# Autodesk Inventor assembly: vehicle assembly v2
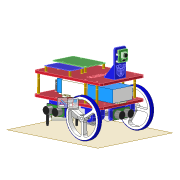
[picture p0: Inventor's stored thumbnail of the model, 180x180]
Saved by Autodesk Inventor 2022 (Build 260153000, 153)
## iProperties
Created: 2024-06-06
Part Number: vehicle assembly v2
Document SubType Name: Assembly
Designer: david
Author: david
## Documents named in this file (29)
- C:\Users\david\OneDrive\Documents\Singapore Polytechnic\SP-RITE\WRO FE 2024 (Repository)\models\vehicle 3D model\vehicle assembly v2.iam
- C:\Users\david\OneDrive\Documents\Singapore Polytechnic\SP-RITE\WRO FE 2024 (Repository)\models\vehicle 3D model\base plate.ipt
- C:\Users\david\OneDrive\Documents\Singapore Polytechnic\SP-RITE\WRO FE 2024 (Repository)\models\vehicle 3D model\bearing holder.ipt
- C:\Users\david\OneDrive\Documents\Singapore Polytechnic\SP-RITE\WRO FE 2024 (Repository)\models\vehicle 3D model\servo motor HS-7955TG.iam
- C:\Users\david\OneDrive\Documents\Singapore Polytechnic\SP-RITE\WRO FE 2024 (Repository)\models\vehicle 3D model\steering top half.ipt
- steering top half.ipt
- C:\Users\david\OneDrive\Documents\Singapore Polytechnic\SP-RITE\WRO FE 2024 (Repository)\models\vehicle 3D model\dfifferential.ipt
- C:\Users\david\OneDrive\Documents\Singapore Polytechnic\SP-RITE\WRO FE 2024 (Repository)\models\vehicle 3D model\front wheel.ipt
- C:\Users\david\OneDrive\Documents\Singapore Polytechnic\SP-RITE\WRO FE 2024 (Repository)\models\vehicle 3D model\rear wheel 86mm.ipt
- C:\Users\david\OneDrive\Documents\Singapore Polytechnic\SP-RITE\WRO FE 2024 (Repository)\models\vehicle 3D model\rear shaft.ipt
- rear shaft.ipt
- C:\Users\david\OneDrive\Documents\Singapore Polytechnic\SP-RITE\WRO FE 2024 (Repository)\models\vehicle 3D model\12v DC motor.ipt
- C:\Users\david\OneDrive\Documents\Singapore Polytechnic\SP-RITE\WRO FE 2024 (Repository)\models\vehicle 3D model\stand M3-L10.ipt
- C:\Users\david\OneDrive\Documents\Singapore Polytechnic\SP-RITE\WRO FE 2024 (Repository)\models\vehicle 3D model\top plate.ipt
- C:\Users\david\OneDrive\Documents\Singapore Polytechnic\SP-RITE\WRO FE 2024 (Repository)\models\vehicle 3D model\raspberry pi.ipt
- C:\Users\david\OneDrive\Documents\Singapore Polytechnic\SP-RITE\WRO FE 2024 (Repository)\models\vehicle 3D model\3s lipo battery.ipt
- C:\Users\david\OneDrive\Documents\Singapore Polytechnic\SP-RITE\WRO FE 2024 (Repository)\models\vehicle 3D model\ultrasonic mount.ipt
- C:\Users\david\OneDrive\Documents\Singapore Polytechnic\SP-RITE\WRO FE 2024 (Repository)\models\vehicle 3D model\US-015.ipt
- C:\Users\david\OneDrive\Documents\Singapore Polytechnic\SP-RITE\WRO FE 2024 (Repository)\models\vehicle 3D model\stand M3-L30.ipt
- C:\Users\david\OneDrive\Documents\Singapore Polytechnic\SP-RITE\WRO FE 2024 (Repository)\models\vehicle 3D model\LM2596 Buck Converter.ipt
- C:\Users\david\OneDrive\Documents\Singapore Polytechnic\SP-RITE\WRO FE 2024 (Repository)\models\vehicle 3D model\camera mount.ipt
- C:\Users\david\OneDrive\Documents\Singapore Polytechnic\SP-RITE\WRO FE 2024 (Repository)\models\vehicle 3D model\raspberry pi camera.ipt
- C:\Users\david\OneDrive\Documents\Singapore Polytechnic\SP-RITE\WRO FE 2024 (Repository)\models\vehicle 3D model\stub.ipt
- C:\Users\david\OneDrive\Documents\Singapore Polytechnic\SP-RITE\WRO FE 2024 (Repository)\models\vehicle 3D model\front shaft.ipt
- C:\Users\david\OneDrive\Documents\Singapore Polytechnic\SP-RITE\WRO FE 2024 (Repository)\models\vehicle 3D model\steering bottom half.ipt
- C:\Users\david\OneDrive\Documents\Singapore Polytechnic\SP-RITE\WRO FE 2024 (Repository)\models\vehicle 3D model\driver gear adapter v2.ipt
- C:\Users\david\OneDrive\Documents\Singapore Polytechnic\SP-RITE\WRO FE 2024 (Repository)\models\vehicle 3D model\ultrasonic mount (front) v2.ipt
- C:\Users\david\OneDrive\Documents\Singapore Polytechnic\SP-RITE\WRO FE 2024 (Repository)\models\vehicle 3D model\3S lipo holder v2.ipt
- C:\Users\david\OneDrive\Documents\Singapore Polytechnic\SP-RITE\WRO FE 2024 (Repository)\models\vehicle 3D model\12v DC motor mount v2.ipt
## Components (56 placed, 26 different names)
1. base plate:1 — Insert:60, Insert:61, Insert:62, Insert:63, Mate:9, Mate:10, Mate:11, Flush:6, Flush:7, Flush:8, Insert:74, Insert:75, Insert:134, Insert:135, Insert:136, Insert:137, Insert:138, Insert:139, Insert:140, Insert:141, Insert:196, Insert:197, Insert:198, Insert:199, Insert:200, Insert:201, Insert:202, Insert:203, Mate:19, Insert:208, Insert:209
2. top plate:1 — Insert:153, Insert:175, Insert:176, Insert:177, Insert:186, Insert:187, Insert:188, Insert:189, Insert:190, Insert:191
3. bearing holder:1 — Insert:134, Insert:135, Insert:143
4. bearing holder:2 — Insert:136, Insert:137
5. bearing holder:3 — Insert:140, Insert:141
6. bearing holder:4 — Insert:138, Insert:139, Insert:142
7. dfifferential:1 — Mate:16, Flush:10
8. rear shaft:1 — Insert:83, Angle:9, Insert:143, Mate:16
9. rear shaft:2 — Angle:8, Insert:142, Insert:205
10. rear wheel 86mm:1 — Insert:83, Angle:9
11. rear wheel 86mm:2 — Tangent:1, Angle:8, Insert:205
12. 12v DC motor:1 — Angle:14, Insert:204, Insert:206, Insert:207
13. servo motor HS-7955TG:1 [sub-assembly] — Mate:2, Insert:20, Mate:9, Mate:10, Mate:11
14. steering top half:1 — Insert:20, Mate:14, Mate:15, Angle:12, Angle:13
15. steering bottom half:1 — Mate:14, Mate:15, Angle:12, Insert:166
16. front wheel:1 — Insert:164, Angle:10
17. front wheel:2 — Insert:165, Angle:11
18. stand M3-L30:2 — Insert:60, Insert:150
19. stand M3-L30:3 — Insert:63, Insert:146
20. stand M3-L30:1 — Insert:61, Insert:151
21. stand M3-L30:4 — Insert:62, Insert:148
22. stand M3-L30:9 — Insert:74, Insert:149
23. stand M3-L30:10 — Insert:75, Insert:147
24. stand M3-L10:1 — Insert:169, Insert:191
25. stand M3-L10:2 — Insert:168, Insert:189
26. stand M3-L10:3 — Insert:59
27. stand M3-L10:4 — Insert:58
28. 3s lipo battery:1 — Flush:9, Mate:18, Flush:11
29. ultrasonic mount:1 — Insert:102, Insert:103, Insert:200, Insert:201
30. ultrasonic mount:2 — Insert:106, Insert:107, Insert:198, Insert:199
31. US-015:1 — Insert:102, Insert:103
32. US-015:2 — Insert:106, Insert:107
33. US-015:3 — Insert:194, Insert:195
34. LM2596 Buck Converter:1 — Insert:112, Insert:113, Insert:169, Insert:170
35. stand M3-L10:5 — Insert:167, Insert:188
36. stand M3-L10:6 — Insert:170, Insert:190
37. stand M3-L10:7 — Insert:112
38. stand M3-L10:8 — Insert:113
39. raspberry pi:1 — Insert:58, Insert:59, Insert:167, Insert:168
40. camera mount:1 — Insert:124, Insert:125, Insert:186, Insert:187
41. raspberry pi camera:1 — Insert:120, Insert:121, Insert:122, Insert:123
42. stub:1 — Insert:123
43. stub:2 — Insert:121, Insert:124
44. stub:3 — Insert:122
45. stub:4 — Insert:120, Insert:125
46. stand M3-L10:9 — Insert:148, Insert:177
47. stand M3-L10:10 — Insert:147
48. stand M3-L10:11 — Insert:151, Insert:153
49. stand M3-L10:12 — Insert:150, Insert:175
50. stand M3-L10:13 — Insert:149
51. stand M3-L10:14 — Insert:146, Insert:176
52. front shaft — Insert:164, Angle:10, Insert:165, Angle:11, Insert:166
53. driver gear adapter v2:1 — Angle:14, Insert:204
54. ultrasonic mount (front) v2:1 — Insert:194, Insert:195, Insert:196, Insert:197
55. 3S lipo holder v2:1 — Insert:202, Insert:203, Mate:18, Flush:11
56. 12v DC motor mount v2:1 — Mate:19, Insert:206, Insert:207, Insert:208, Insert:209
## Relationships (95: Insert 71, Mate 9, Angle 8, Flush 6, Tangent 1)
- Mate:2: servo motor HS-7955TG:1
- Insert:20: servo motor HS-7955TG:1 ↔ steering top half:1
- Angle:4 (0 deg)
- Tangent:1: rear wheel 86mm:2
- Insert:58: stand M3-L10:4 ↔ raspberry pi:1
- Insert:59: stand M3-L10:3 ↔ raspberry pi:1
- Insert:60: base plate:1 ↔ stand M3-L30:2
- Insert:61: base plate:1 ↔ stand M3-L30:1
- Insert:62: base plate:1 ↔ stand M3-L30:4
- Insert:63: base plate:1 ↔ stand M3-L30:3
- Mate:9: base plate:1 ↔ servo motor HS-7955TG:1
- Mate:10: base plate:1 ↔ servo motor HS-7955TG:1
- Mate:11: base plate:1 ↔ servo motor HS-7955TG:1
- Flush:6: base plate:1
- Flush:7: base plate:1
- Flush:8: base plate:1
- Insert:74: base plate:1 ↔ stand M3-L30:9
- Insert:75: base plate:1 ↔ stand M3-L30:10
- Insert:83: rear shaft:1 ↔ rear wheel 86mm:1
- Angle:8 (180 deg): rear shaft:2 ↔ rear wheel 86mm:2
- Angle:9 (180 deg): rear shaft:1 ↔ rear wheel 86mm:1
- Insert:102: ultrasonic mount:1 ↔ US-015:1
- Insert:103: ultrasonic mount:1 ↔ US-015:1
- Insert:106: ultrasonic mount:2 ↔ US-015:2
- Insert:107: ultrasonic mount:2 ↔ US-015:2
- Insert:112: LM2596 Buck Converter:1 ↔ stand M3-L10:7
- Insert:113: LM2596 Buck Converter:1 ↔ stand M3-L10:8
- Insert:120: raspberry pi camera:1 ↔ stub:4
- Insert:121: raspberry pi camera:1 ↔ stub:2
- Insert:122: raspberry pi camera:1 ↔ stub:3
- Insert:123: raspberry pi camera:1 ↔ stub:1
- Insert:124: camera mount:1 ↔ stub:2
- Insert:125: camera mount:1 ↔ stub:4
- Insert:134: base plate:1 ↔ bearing holder:1
- Insert:135: base plate:1 ↔ bearing holder:1
- Insert:136: base plate:1 ↔ bearing holder:2
- Insert:137: base plate:1 ↔ bearing holder:2
- Insert:138: base plate:1 ↔ bearing holder:4
- Insert:139: base plate:1 ↔ bearing holder:4
- Insert:140: base plate:1 ↔ bearing holder:3
- Insert:141: base plate:1 ↔ bearing holder:3
- Insert:142: bearing holder:4 ↔ rear shaft:2
- Insert:143: bearing holder:1 ↔ rear shaft:1
- Insert:146: stand M3-L30:3 ↔ stand M3-L10:14
- Insert:147: stand M3-L30:10 ↔ stand M3-L10:10
- Insert:148: stand M3-L30:4 ↔ stand M3-L10:9
- Insert:149: stand M3-L30:9 ↔ stand M3-L10:13
- Insert:150: stand M3-L30:2 ↔ stand M3-L10:12
- Insert:151: stand M3-L30:1 ↔ stand M3-L10:11
- Insert:153: top plate:1 ↔ stand M3-L10:11
- Flush:9: 3s lipo battery:1
- Insert:164: front wheel:1 ↔ front shaft
- Angle:10 (0 deg): front wheel:1 ↔ front shaft
- Insert:165: front wheel:2 ↔ front shaft
- Angle:11 (0 deg): front wheel:2 ↔ front shaft
- Mate:14: steering top half:1 ↔ steering bottom half:1
- Mate:15: steering top half:1 ↔ steering bottom half:1
- Angle:12 (180 deg): steering top half:1 ↔ steering bottom half:1
- Insert:166: steering bottom half:1 ↔ front shaft
- Angle:13 (45 deg): steering top half:1
- Insert:167: stand M3-L10:5 ↔ raspberry pi:1
- Insert:168: stand M3-L10:2 ↔ raspberry pi:1
- Insert:169: stand M3-L10:1 ↔ LM2596 Buck Converter:1
- Insert:170: LM2596 Buck Converter:1 ↔ stand M3-L10:6
- Insert:175: top plate:1 ↔ stand M3-L10:12
- Insert:176: top plate:1 ↔ stand M3-L10:14
- Insert:177: top plate:1 ↔ stand M3-L10:9
- Mate:16: dfifferential:1 ↔ rear shaft:1
- Flush:10: dfifferential:1
- Insert:186: top plate:1 ↔ camera mount:1
- Insert:187: top plate:1 ↔ camera mount:1
- Insert:188: top plate:1 ↔ stand M3-L10:5
- Insert:189: top plate:1 ↔ stand M3-L10:2
- Insert:190: top plate:1 ↔ stand M3-L10:6
- Insert:191: top plate:1 ↔ stand M3-L10:1
- Insert:194: US-015:3 ↔ ultrasonic mount (front) v2:1
- Insert:195: US-015:3 ↔ ultrasonic mount (front) v2:1
- Insert:196: base plate:1 ↔ ultrasonic mount (front) v2:1
- Insert:197: base plate:1 ↔ ultrasonic mount (front) v2:1
- Insert:198: base plate:1 ↔ ultrasonic mount:2
- Insert:199: base plate:1 ↔ ultrasonic mount:2
- Insert:200: base plate:1 ↔ ultrasonic mount:1
- Insert:201: base plate:1 ↔ ultrasonic mount:1
- Insert:202: base plate:1 ↔ 3S lipo holder v2:1
- Insert:203: base plate:1 ↔ 3S lipo holder v2:1
- Mate:18: 3s lipo battery:1 ↔ 3S lipo holder v2:1
- Angle:14 (180 deg): 12v DC motor:1 ↔ driver gear adapter v2:1
- Insert:204: 12v DC motor:1 ↔ driver gear adapter v2:1
- Flush:11: 3s lipo battery:1 ↔ 3S lipo holder v2:1
- Insert:205: rear shaft:2 ↔ rear wheel 86mm:2
- Mate:19: base plate:1 ↔ 12v DC motor mount v2:1
- Insert:206: 12v DC motor:1 ↔ 12v DC motor mount v2:1
- Insert:207: 12v DC motor:1 ↔ 12v DC motor mount v2:1
- Insert:208: base plate:1 ↔ 12v DC motor mount v2:1
- Insert:209: base plate:1 ↔ 12v DC motor mount v2:1
